# Autodesk Inventor assembly: Power-Reg
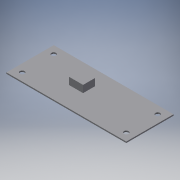
[picture p0: Inventor's stored thumbnail of the model, 180x180]
Saved by Autodesk Inventor 2018 (Build 220112000, 112)
## iProperties
Created: 2018-04-09
Part Number: Power-Reg
Document SubType Name: Assembly
Designer: bbramman
Author: bbramman
## Documents named in this file (3)
- C:\Users\bbramman\OneDrive\Documents\Trapped Ion Research (Grad)\Electronics\pll-evalboard-synthesizer\Box CAD\Power-Reg.iam
- C:\Users\bbramman\OneDrive\Documents\Trapped Ion Research (Grad)\Electronics\pll-evalboard-synthesizer\Box CAD\76x30mm-PCB.ipt
- C:\Users\bbramman\OneDrive\Documents\Trapped Ion Research (Grad)\Electronics\pll-evalboard-synthesizer\Box CAD\Regulator-LT1965.ipt
## Components (2 placed, 2 different names)
1. 76x30mm-PCB:1 — Mate:1
2. Regulator-LT1965:1 — Mate:1
## Relationships (1: Mate 1)
- Mate:1: 76x30mm-PCB:1 ↔ Regulator-LT1965:1
